# Autodesk Inventor assembly: Designtraining_gearbox_3
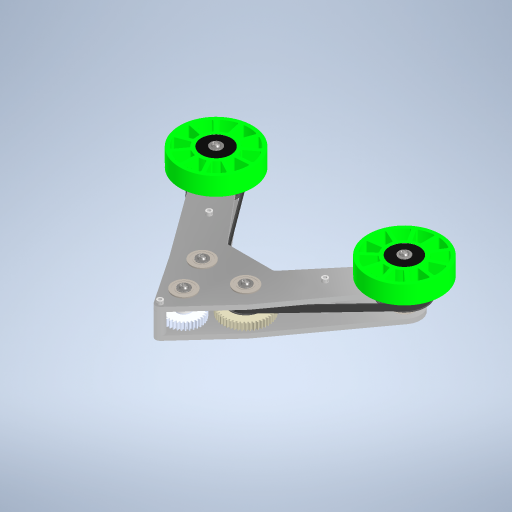
[picture p0: Inventor's stored thumbnail of the model, 512x512]
Saved by Autodesk Inventor 2024 (Build 280153000, 153)
## iProperties
Created: 2024-12-21
Part Number: Designtraining_gearbox_3
Document SubType Name: Assembly
Designer: Danielle
Author: Danielle
## Documents named in this file (19)
- C:\Users\micha\OneDrive\Documents\GitHub\1622-2024-Assignments\Danielle\gearbox 3\Designtraining_gearbox_3.iam
- C:\Users\micha\OneDrive\Documents\bottomplate_gearbox3_.ipt
- C:\Users\micha\OneDrive\Documents\topplate_gearbox3_.ipt
- C:\Users\micha\OneDrive\Documents\GitHub\1622-2024-Assignments\COTS Library\Motion\Gears\20DP gears\Aluminum\COTS_WCP-0188.ipt
- C:\Users\micha\OneDrive\Documents\GitHub\1622-2024-Assignments\Danielle\gearbox 3\gearbox 3 stuff\WCP-0709\WCP-0709.ipt
- C:\Users\micha\OneDrive\Documents\GitHub\1622-2024-Assignments\Danielle\gearbox 3\gearbox 3 stuff\WCP-0783\WCP-0783.ipt
- C:\Users\micha\OneDrive\Documents\GitHub\1622-2024-Assignments\Danielle\gearbox 3\gearbox 3 stuff\WCP-0564\WCP-0564.ipt
- C:\Users\micha\OneDrive\Documents\GitHub\1622-2024-Assignments\Danielle\gearbox 3\gearbox 3 stuff\WCP-0990\WCP-0990.ipt
- C:\Users\micha\OneDrive\Documents\GitHub\1622-2024-Assignments\Danielle\gearbox 3\gearbox 3 stuff too\acetalspacer.ipt
- C:\Users\micha\OneDrive\Documents\GitHub\1622-2024-Assignments\Danielle\gearbox 3\gearbox 3 stuff too\standoff_1.131inches.ipt
- C:\Users\micha\OneDrive\Documents\GitHub\1622-2024-Assignments\Danielle\gearbox 3\gearbox 3 stuff too\spacer_0.498inches.ipt
- C:\Users\micha\OneDrive\Documents\GitHub\1622-2024-Assignments\Danielle\gearbox 3\gearbox 3 stuff too\spacer_0.633inches.ipt
- C:\Users\micha\OneDrive\Documents\GitHub\1622-2024-Assignments\Danielle\gearbox 3\gearbox 3 stuff too\1.756in_hexshaft.ipt
- C:\Users\micha\OneDrive\Documents\GitHub\1622-2024-Assignments\COTS Library\Motion\Wheels\Compliant Wheels\4in compliant wheels\0.500in hex bore\COTS_am-3462_4indiameter_0.500inhexbore_durometer35A_CompliantWheel.ipt
- C:\Users\micha\OneDrive\Documents\GitHub\1622-2024-Assignments\Danielle\gearbox 3\gearbox 3 stuff too\2.756_hexshaft.ipt
- C:\Users\micha\OneDrive\Documents\GitHub\1622-2024-Assignments\Danielle\gearbox 2\gearbox 2 stuff\92949A535_18-8 Stainless Steel Button Head Hex Drive Screw (1)\92949A535_18-8 Stainless Steel Button Head Hex Dr.ipt
- C:\Users\micha\OneDrive\Documents\GitHub\1622-2024-Assignments\Danielle\gearbox 2\gearbox 2 stuff\90107A029_316 Stainless Steel Washer\90107A029_316 Stainless Steel Washer.ipt
- C:\Users\micha\OneDrive\Documents\GitHub\1622-2024-Assignments\Danielle\gearbox 3\gearbox 3 stuff\91251A352_Black-Oxide Alloy Steel Socket Head Screw\91251A352_Black-Oxide Alloy Steel Socket Head Screw.ipt
- C:\Users\micha\OneDrive\Documents\GitHub\1622-2024-Assignments\Danielle\gearbox 3\gearbox 3 stuff too\9mm_belt.ipt
## Components (61 placed, 18 different names)
1. bottomplate_gearbox3_:1 — Mate:1, Mate:2, Mate:3, Mate:4, Mate:5, Mate:6, Mate:7, Mate:18, Mate:19, Mate:20, Mate:21, Mate:22, Mate:23, Mate:24, Mate:25, Mate:26, Mate:27, Mate:47, Mate:49, Mate:51
2. topplate_gearbox3_:1 — Mate:1, Mate:2, Mate:8, Mate:9, Mate:10, Mate:11, Mate:12, Mate:13, Mate:14, Mate:15, Mate:16, Mate:17, Mate:48, Mate:50, Mate:52, Mate:58, Mate:118, Mate:119, Mate:120, Mate:121, Mate:122, Mate:123
3. COTS_WCP-0188:1 — Mate:28, Flush:1, Mate:30, Mate:35, Mate:37, Angle:6, Angle:7
4. WCP-0709:1 — Mate:31, Mate:32, Angle:10, Angle:11, Mate:59
5. COTS_WCP-0188:2 — Mate:29, Flush:1, Mate:36, Angle:12, Angle:13
6. WCP-0783:1 — Mate:12, Mate:13, Mate:46, Angle:19, Mate:66, Mate:67
7. WCP-0783:2 — Mate:11, Mate:14, Angle:15, Mate:63, Angle:23, Flush:7
8. WCP-0783:3 — Mate:10, Mate:15, Angle:11, Mate:60, Angle:20, Mate:61, Angle:21, Flush:5
9. WCP-0783:4 — Mate:9, Mate:16, Angle:9, Mate:62, Angle:22, Flush:6, Mate:105
10. WCP-0783:5 — Mate:8, Mate:17, Angle:4, Mate:57, Mate:64, Mate:65
11. WCP-0783:6 — Mate:22, Mate:27, Mate:34, Mate:53, Angle:16
12. WCP-0783:7 — Mate:21, Mate:26, Mate:29, Angle:12
13. WCP-0783:8 — Mate:20, Mate:25, Mate:31, Mate:32, Angle:10
14. WCP-0783:9 — Mate:19, Mate:24, Mate:28, Mate:30, Angle:6
15. WCP-0783:10 — Mate:18, Mate:23, Mate:33, Mate:55, Angle:1
16. WCP-0564:1 — Mate:36, Flush:2, Flush:4, Mate:41, Mate:44, Angle:13, Angle:14, Mate:124, Mate:125
17. WCP-0990:1 — Mate:33, Flush:3, Mate:56, Angle:2, Angle:4, Angle:5, Angle:24, Mate:129
18. WCP-0564:2 — Mate:35, Flush:2, Mate:37, Flush:3, Mate:40, Mate:43, Angle:7, Angle:8, Mate:127, Mate:128
19. WCP-0990:2 — Mate:34, Flush:4, Mate:42, Mate:45, Mate:54, Angle:17, Angle:18, Angle:25, Mate:126
20. acetalspacer:2 — Mate:40, Mate:43, Angle:8, Angle:9
21. acetalspacer:3 — Mate:41, Mate:44, Angle:14, Angle:15
22. acetalspacer:4 — Mate:42, Mate:45, Mate:46, Angle:18, Angle:19
23. standoff_1.131inches:1 — Mate:51, Mate:52
24. standoff_1.131inches:2 — Mate:47, Mate:48
25. standoff_1.131inches:3 — Mate:49, Mate:50
26. spacer_0.498inches:1 — Mate:53, Mate:54, Angle:16, Angle:17
27. spacer_0.498inches:2 — Mate:55, Mate:56, Angle:1, Angle:2
28. acetalspacer:5 — Mate:57, Mate:58, Angle:5
29. spacer_0.633inches:1 — Mate:59, Mate:60, Angle:20
30. 1.756in_hexshaft:1 — Mate:63, Angle:23, Flush:7, Mate:98, Mate:99, Mate:110, Mate:114
31. 1.756in_hexshaft:2 — Mate:61, Angle:21, Flush:5, Mate:100, Mate:106, Mate:109, Mate:115
32. 1.756in_hexshaft:3 — Mate:62, Angle:22, Flush:6, Mate:101, Mate:111, Mate:116
33. COTS_am-3462_4indiameter_0.500inhexbore_durometer35A_CompliantWheel:1 — Mate:64, Mate:65, Angle:24, Mate:69, Angle:27, Flush:9
34. COTS_am-3462_4indiameter_0.500inhexbore_durometer35A_CompliantWheel:2 — Mate:66, Mate:67, Angle:25, Mate:68, Angle:26, Flush:8
35. 2.756_hexshaft:1 — Mate:69, Angle:27, Flush:9, Mate:103, Mate:107, Mate:112, Mate:117
36. 2.756_hexshaft:2 — Mate:68, Angle:26, Flush:8, Mate:102, Mate:104, Mate:108, Mate:113
37. 92949A535_18-8 Stainless Steel Button Head Hex Dr:10 — Mate:77, Mate:79, Mate:98
38. 90107A029_316 Stainless Steel Washer:8 — Mate:77, Mate:79, Mate:99
39. 92949A535_18-8 Stainless Steel Button Head Hex Dr:11 — Mate:110
40. 90107A029_316 Stainless Steel Washer:9 — Mate:114
41. 92949A535_18-8 Stainless Steel Button Head Hex Dr:12 — Mate:101
42. 90107A029_316 Stainless Steel Washer:10 — Mate:105
43. 92949A535_18-8 Stainless Steel Button Head Hex Dr:13 — Mate:108
44. 90107A029_316 Stainless Steel Washer:11 — Mate:113
45. 92949A535_18-8 Stainless Steel Button Head Hex Dr:14 — Mate:109
46. 90107A029_316 Stainless Steel Washer:12 — Mate:115
47. 92949A535_18-8 Stainless Steel Button Head Hex Dr:15 — Mate:112
48. 90107A029_316 Stainless Steel Washer:13 — Mate:117
49. 92949A535_18-8 Stainless Steel Button Head Hex Dr:16 — Mate:111
50. 90107A029_316 Stainless Steel Washer:14 — Mate:116
51. 92949A535_18-8 Stainless Steel Button Head Hex Dr:17 — Mate:103
52. 90107A029_316 Stainless Steel Washer:15 — Mate:107
53. 92949A535_18-8 Stainless Steel Button Head Hex Dr:18 — Mate:100
54. 90107A029_316 Stainless Steel Washer:16 — Mate:106
55. 92949A535_18-8 Stainless Steel Button Head Hex Dr:19 — Mate:102
56. 90107A029_316 Stainless Steel Washer:17 — Mate:104
57. 91251A352_Black-Oxide Alloy Steel Socket Head Screw:1 — Mate:119, Mate:123
58. 91251A352_Black-Oxide Alloy Steel Socket Head Screw:2 — Mate:120, Mate:122
59. 91251A352_Black-Oxide Alloy Steel Socket Head Screw:3 — Mate:118, Mate:121
60. 9mm_belt:1 — Mate:124, Mate:125, Mate:126
61. 9mm_belt:2 — Mate:127, Mate:128, Mate:129
## Relationships (154: Mate 119, Angle 26, Flush 9)
- Mate:1: bottomplate_gearbox3_:1 ↔ topplate_gearbox3_:1
- Mate:2: bottomplate_gearbox3_:1 ↔ topplate_gearbox3_:1
- Mate:3: bottomplate_gearbox3_:1
- Mate:4: bottomplate_gearbox3_:1
- Mate:5: bottomplate_gearbox3_:1
- Mate:6: bottomplate_gearbox3_:1
- Mate:7: bottomplate_gearbox3_:1
- Mate:8: topplate_gearbox3_:1 ↔ WCP-0783:5
- Mate:9: topplate_gearbox3_:1 ↔ WCP-0783:4
- Mate:10: topplate_gearbox3_:1 ↔ WCP-0783:3
- Mate:11: topplate_gearbox3_:1 ↔ WCP-0783:2
- Mate:12: topplate_gearbox3_:1 ↔ WCP-0783:1
- Mate:13: topplate_gearbox3_:1 ↔ WCP-0783:1
- Mate:14: topplate_gearbox3_:1 ↔ WCP-0783:2
- Mate:15: topplate_gearbox3_:1 ↔ WCP-0783:3
- Mate:16: topplate_gearbox3_:1 ↔ WCP-0783:4
- Mate:17: topplate_gearbox3_:1 ↔ WCP-0783:5
- Mate:18: bottomplate_gearbox3_:1 ↔ WCP-0783:10
- Mate:19: bottomplate_gearbox3_:1 ↔ WCP-0783:9
- Mate:20: bottomplate_gearbox3_:1 ↔ WCP-0783:8
- Mate:21: bottomplate_gearbox3_:1 ↔ WCP-0783:7
- Mate:22: bottomplate_gearbox3_:1 ↔ WCP-0783:6
- Mate:23: bottomplate_gearbox3_:1 ↔ WCP-0783:10
- Mate:24: bottomplate_gearbox3_:1 ↔ WCP-0783:9
- Mate:25: bottomplate_gearbox3_:1 ↔ WCP-0783:8
- Mate:26: bottomplate_gearbox3_:1 ↔ WCP-0783:7
- Mate:27: bottomplate_gearbox3_:1 ↔ WCP-0783:6
- Mate:28: COTS_WCP-0188:1 ↔ WCP-0783:9
- Mate:29: COTS_WCP-0188:2 ↔ WCP-0783:7
- Flush:1: COTS_WCP-0188:1 ↔ COTS_WCP-0188:2
- Mate:30: COTS_WCP-0188:1 ↔ WCP-0783:9
- Mate:31: WCP-0709:1 ↔ WCP-0783:8
- Mate:32: WCP-0709:1 ↔ WCP-0783:8
- Mate:33: WCP-0783:10 ↔ WCP-0990:1
- Mate:34: WCP-0783:6 ↔ WCP-0990:2
- Mate:35: COTS_WCP-0188:1 ↔ WCP-0564:2
- Mate:36: COTS_WCP-0188:2 ↔ WCP-0564:1
- Flush:2: WCP-0564:1 ↔ WCP-0564:2
- Mate:37: COTS_WCP-0188:1 ↔ WCP-0564:2
- Flush:3: WCP-0990:1 ↔ WCP-0564:2
- Flush:4: WCP-0564:1 ↔ WCP-0990:2
- Mate:40: WCP-0564:2 ↔ acetalspacer:2
- Mate:41: WCP-0564:1 ↔ acetalspacer:3
- Mate:42: WCP-0990:2 ↔ acetalspacer:4
- Mate:43: WCP-0564:2 ↔ acetalspacer:2
- Mate:44: WCP-0564:1 ↔ acetalspacer:3
- Mate:45: WCP-0990:2 ↔ acetalspacer:4
- Mate:46: WCP-0783:1 ↔ acetalspacer:4
- Mate:47: bottomplate_gearbox3_:1 ↔ standoff_1.131inches:2
- Mate:48: topplate_gearbox3_:1 ↔ standoff_1.131inches:2
- Mate:49: bottomplate_gearbox3_:1 ↔ standoff_1.131inches:3
- Mate:50: topplate_gearbox3_:1 ↔ standoff_1.131inches:3
- Mate:51: bottomplate_gearbox3_:1 ↔ standoff_1.131inches:1
- Mate:52: topplate_gearbox3_:1 ↔ standoff_1.131inches:1
- Mate:53: WCP-0783:6 ↔ spacer_0.498inches:1
- Mate:54: WCP-0990:2 ↔ spacer_0.498inches:1
- Mate:55: WCP-0783:10 ↔ spacer_0.498inches:2
- Mate:56: WCP-0990:1 ↔ spacer_0.498inches:2
- Angle:1 (0 deg): WCP-0783:10 ↔ spacer_0.498inches:2
- Angle:2 (0 deg): WCP-0990:1 ↔ spacer_0.498inches:2
- Angle:4 (0 deg): WCP-0783:5 ↔ WCP-0990:1
- Mate:57: WCP-0783:5 ↔ acetalspacer:5
- Mate:58: topplate_gearbox3_:1 ↔ acetalspacer:5
- Angle:5 (0 deg): WCP-0990:1 ↔ acetalspacer:5
- Angle:6 (0 deg): COTS_WCP-0188:1 ↔ WCP-0783:9
- Angle:7 (0 deg): COTS_WCP-0188:1 ↔ WCP-0564:2
- Angle:8 (0 deg): WCP-0564:2 ↔ acetalspacer:2
- Angle:9 (0 deg): WCP-0783:4 ↔ acetalspacer:2
- Angle:10 (0 deg): WCP-0709:1 ↔ WCP-0783:8
- Angle:11 (0 deg): WCP-0709:1 ↔ WCP-0783:3
- Angle:12 (0 deg): COTS_WCP-0188:2 ↔ WCP-0783:7
- Angle:13 (0 deg): COTS_WCP-0188:2 ↔ WCP-0564:1
- Angle:14 (0 deg): WCP-0564:1 ↔ acetalspacer:3
- Angle:15 (0 deg): WCP-0783:2 ↔ acetalspacer:3
- Angle:16 (0 deg): WCP-0783:6 ↔ spacer_0.498inches:1
- Angle:17 (0 deg): WCP-0990:2 ↔ spacer_0.498inches:1
- Angle:18 (0 deg): WCP-0990:2 ↔ acetalspacer:4
- Angle:19 (0 deg): WCP-0783:1 ↔ acetalspacer:4
- Mate:59: WCP-0709:1 ↔ spacer_0.633inches:1
- Mate:60: WCP-0783:3 ↔ spacer_0.633inches:1
- Angle:20 (0 deg): WCP-0783:3 ↔ spacer_0.633inches:1
- Mate:61: WCP-0783:3 ↔ 1.756in_hexshaft:2
- Angle:21 (0 deg): WCP-0783:3 ↔ 1.756in_hexshaft:2
- Flush:5: WCP-0783:3 ↔ 1.756in_hexshaft:2
- Mate:62: WCP-0783:4 ↔ 1.756in_hexshaft:3
- Angle:22 (0 deg): WCP-0783:4 ↔ 1.756in_hexshaft:3
- Flush:6: WCP-0783:4 ↔ 1.756in_hexshaft:3
- Mate:63: WCP-0783:2 ↔ 1.756in_hexshaft:1
- Angle:23 (0 deg): WCP-0783:2 ↔ 1.756in_hexshaft:1
- Flush:7: WCP-0783:2 ↔ 1.756in_hexshaft:1
- Mate:64: WCP-0783:5 ↔ COTS_am-3462_4indiameter_0.500inhexbore_durometer35A_CompliantWheel:1
- Mate:65: WCP-0783:5 ↔ COTS_am-3462_4indiameter_0.500inhexbore_durometer35A_CompliantWheel:1
- Mate:66: WCP-0783:1 ↔ COTS_am-3462_4indiameter_0.500inhexbore_durometer35A_CompliantWheel:2
- Mate:67: WCP-0783:1 ↔ COTS_am-3462_4indiameter_0.500inhexbore_durometer35A_CompliantWheel:2
- Angle:24 (0 deg): WCP-0990:1 ↔ COTS_am-3462_4indiameter_0.500inhexbore_durometer35A_CompliantWheel:1
- Angle:25 (0 deg): WCP-0990:2 ↔ COTS_am-3462_4indiameter_0.500inhexbore_durometer35A_CompliantWheel:2
- Mate:68: COTS_am-3462_4indiameter_0.500inhexbore_durometer35A_CompliantWheel:2 ↔ 2.756_hexshaft:2
- Angle:26 (0 deg): COTS_am-3462_4indiameter_0.500inhexbore_durometer35A_CompliantWheel:2 ↔ 2.756_hexshaft:2
- Flush:8: COTS_am-3462_4indiameter_0.500inhexbore_durometer35A_CompliantWheel:2 ↔ 2.756_hexshaft:2
- Mate:69: COTS_am-3462_4indiameter_0.500inhexbore_durometer35A_CompliantWheel:1 ↔ 2.756_hexshaft:1
- Angle:27 (0 deg): COTS_am-3462_4indiameter_0.500inhexbore_durometer35A_CompliantWheel:1 ↔ 2.756_hexshaft:1
- Flush:9: COTS_am-3462_4indiameter_0.500inhexbore_durometer35A_CompliantWheel:1 ↔ 2.756_hexshaft:1
- Mate:77: 92949A535_18-8 Stainless Steel Button Head Hex Dr:10 ↔ 90107A029_316 Stainless Steel Washer:8
- Mate:79: 92949A535_18-8 Stainless Steel Button Head Hex Dr:10 ↔ 90107A029_316 Stainless Steel Washer:8
- [Mate]: 92949A535_18-8 Stainless Steel Button Head Hex Dr:11 ↔ 90107A029_316 Stainless Steel Washer:9
- [Mate]: 92949A535_18-8 Stainless Steel Button Head Hex Dr:11 ↔ 90107A029_316 Stainless Steel Washer:9
- [Mate]: 92949A535_18-8 Stainless Steel Button Head Hex Dr:12 ↔ 90107A029_316 Stainless Steel Washer:10
- [Mate]: 92949A535_18-8 Stainless Steel Button Head Hex Dr:12 ↔ 90107A029_316 Stainless Steel Washer:10
- [Mate]: 92949A535_18-8 Stainless Steel Button Head Hex Dr:13 ↔ 90107A029_316 Stainless Steel Washer:11
- [Mate]: 92949A535_18-8 Stainless Steel Button Head Hex Dr:13 ↔ 90107A029_316 Stainless Steel Washer:11
- [Mate]: 92949A535_18-8 Stainless Steel Button Head Hex Dr:14 ↔ 90107A029_316 Stainless Steel Washer:12
- [Mate]: 92949A535_18-8 Stainless Steel Button Head Hex Dr:14 ↔ 90107A029_316 Stainless Steel Washer:12
- [Mate]: 92949A535_18-8 Stainless Steel Button Head Hex Dr:15 ↔ 90107A029_316 Stainless Steel Washer:13
- [Mate]: 92949A535_18-8 Stainless Steel Button Head Hex Dr:15 ↔ 90107A029_316 Stainless Steel Washer:13
- [Mate]: 92949A535_18-8 Stainless Steel Button Head Hex Dr:16 ↔ 90107A029_316 Stainless Steel Washer:14
- [Mate]: 92949A535_18-8 Stainless Steel Button Head Hex Dr:16 ↔ 90107A029_316 Stainless Steel Washer:14
- [Mate]: 92949A535_18-8 Stainless Steel Button Head Hex Dr:17 ↔ 90107A029_316 Stainless Steel Washer:15
- [Mate]: 92949A535_18-8 Stainless Steel Button Head Hex Dr:17 ↔ 90107A029_316 Stainless Steel Washer:15
- [Mate]: 92949A535_18-8 Stainless Steel Button Head Hex Dr:18 ↔ 90107A029_316 Stainless Steel Washer:16
- [Mate]: 92949A535_18-8 Stainless Steel Button Head Hex Dr:18 ↔ 90107A029_316 Stainless Steel Washer:16
- [Mate]: 92949A535_18-8 Stainless Steel Button Head Hex Dr:19 ↔ 90107A029_316 Stainless Steel Washer:17
- [Mate]: 92949A535_18-8 Stainless Steel Button Head Hex Dr:19 ↔ 90107A029_316 Stainless Steel Washer:17
- Mate:98: 1.756in_hexshaft:1 ↔ 92949A535_18-8 Stainless Steel Button Head Hex Dr:10
- Mate:99: 1.756in_hexshaft:1 ↔ 90107A029_316 Stainless Steel Washer:8
- Mate:100: 1.756in_hexshaft:2 ↔ 92949A535_18-8 Stainless Steel Button Head Hex Dr:18
- Mate:101: 1.756in_hexshaft:3 ↔ 92949A535_18-8 Stainless Steel Button Head Hex Dr:12
- Mate:102: 2.756_hexshaft:2 ↔ 92949A535_18-8 Stainless Steel Button Head Hex Dr:19
- Mate:103: 2.756_hexshaft:1 ↔ 92949A535_18-8 Stainless Steel Button Head Hex Dr:17
- Mate:104: 2.756_hexshaft:2 ↔ 90107A029_316 Stainless Steel Washer:17
- Mate:105: WCP-0783:4 ↔ 90107A029_316 Stainless Steel Washer:10
- Mate:106: 1.756in_hexshaft:2 ↔ 90107A029_316 Stainless Steel Washer:16
- Mate:107: 2.756_hexshaft:1 ↔ 90107A029_316 Stainless Steel Washer:15
- Mate:108: 2.756_hexshaft:2 ↔ 92949A535_18-8 Stainless Steel Button Head Hex Dr:13
- Mate:109: 1.756in_hexshaft:2 ↔ 92949A535_18-8 Stainless Steel Button Head Hex Dr:14
- Mate:110: 1.756in_hexshaft:1 ↔ 92949A535_18-8 Stainless Steel Button Head Hex Dr:11
- Mate:111: 1.756in_hexshaft:3 ↔ 92949A535_18-8 Stainless Steel Button Head Hex Dr:16
- Mate:112: 2.756_hexshaft:1 ↔ 92949A535_18-8 Stainless Steel Button Head Hex Dr:15
- Mate:113: 2.756_hexshaft:2 ↔ 90107A029_316 Stainless Steel Washer:11
- Mate:114: 1.756in_hexshaft:1 ↔ 90107A029_316 Stainless Steel Washer:9
- Mate:115: 1.756in_hexshaft:2 ↔ 90107A029_316 Stainless Steel Washer:12
- Mate:116: 1.756in_hexshaft:3 ↔ 90107A029_316 Stainless Steel Washer:14
- Mate:117: 2.756_hexshaft:1 ↔ 90107A029_316 Stainless Steel Washer:13
- Mate:118: topplate_gearbox3_:1 ↔ 91251A352_Black-Oxide Alloy Steel Socket Head Screw:3
- Mate:119: topplate_gearbox3_:1 ↔ 91251A352_Black-Oxide Alloy Steel Socket Head Screw:1
- Mate:120: topplate_gearbox3_:1 ↔ 91251A352_Black-Oxide Alloy Steel Socket Head Screw:2
- Mate:121: topplate_gearbox3_:1 ↔ 91251A352_Black-Oxide Alloy Steel Socket Head Screw:3
- Mate:122: topplate_gearbox3_:1 ↔ 91251A352_Black-Oxide Alloy Steel Socket Head Screw:2
- Mate:123: topplate_gearbox3_:1 ↔ 91251A352_Black-Oxide Alloy Steel Socket Head Screw:1
- Mate:124: WCP-0564:1 ↔ 9mm_belt:1
- Mate:125: WCP-0564:1 ↔ 9mm_belt:1
- Mate:126: WCP-0990:2 ↔ 9mm_belt:1
- Mate:127: WCP-0564:2 ↔ 9mm_belt:2
- Mate:128: WCP-0564:2 ↔ 9mm_belt:2
- Mate:129: WCP-0990:1 ↔ 9mm_belt:2
## Named parameters: d116_d112 = 0 mm, d117_d114 = 0 mm, d118_d112 = 0 mm, d119_d114 = 0 mm, d120_d112 = 0 mm, d121_d114 = 0 mm, d122_d112 = 0 mm, d123_d114 = 0 mm, d124_d112 = 0 mm, d125_d114 = 0 mm, d126_d112 = 0 mm, d127_d114 = 0 mm, d128_d112 = 0 mm, d129_d114 = 0 mm, d130_d112 = 0 mm, d131_d114 = 0 mm, d132_d112 = 0 mm, d133_d114 = 0 mm
